# Autodesk Inventor assembly: CrutchCupHolder
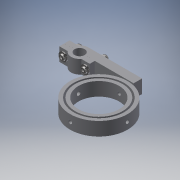
[picture p0: Inventor's stored thumbnail of the model, 180x180]
Saved by Autodesk Inventor 2017 SP1 (Build 210196100, 196)
## iProperties
Created: 2016-07-31
Part Number: CrutchCupHolder
Document SubType Name: Assembly
Designer: steele
Author: steele
## Documents named in this file (8)
- D:\snobotics\CAD-Development\robSteele\HouseProjects\CrutchProjects\CrutchCupHolder.iam
- D:\snobotics\CAD-Development\robSteele\HouseProjects\CrutchProjects\Innerring.ipt
- D:\snobotics\CAD-Development\robSteele\HouseProjects\CrutchProjects\outerRing.ipt
- D:\snobotics\CAD-Development\robSteele\HouseProjects\CrutchProjects\outerCrutchAttacement.ipt
- D:\snobotics\CAD-Development\robSteele\HouseProjects\CrutchProjects\innerCrutchAttacement.ipt
- D:\snobotics\CAD-Development\robSteele\HouseProjects\CrutchProjects\CrutchCupHolder\Design Accelerator\Bolted Connection1.iam
- D:\snobotics\CAD-Development\robSteele\HouseProjects\CrutchProjects\CrutchCupHolder\Design Accelerator\Bolted Connection2.iam
- D:\snobotics\CAD-Development\robSteele\HouseProjects\CrutchProjects\CrutchCupHolder\Design Accelerator\Clevis Pin Connection4.iam
## Components (7 placed, 6 different names)
1. Innerring:1 — Insert:1
2. outerRing:1 — Mate:8, Insert:1
3. outerCrutchAttacement:1 — Mate:1, Flush:1, Flush:2, Mate:9, Mate:10
4. innerCrutchAttacement:1 — Mate:1, Flush:1, Flush:2, Mate:2, Mate:3, Mate:4, Mate:5
5. Bolted Connection:1 [sub-assembly] — Mate:2, Mate:3
6. Bolted Connection:2 [sub-assembly] — Mate:4, Mate:5
7. Clevis Pin Connection:1 [sub-assembly] — Mate:8, Mate:9, Mate:10
## Relationships (11: Mate 8, Flush 2, Insert 1)
- Mate:1: outerCrutchAttacement:1 ↔ innerCrutchAttacement:1
- Flush:1: outerCrutchAttacement:1 ↔ innerCrutchAttacement:1
- Flush:2: outerCrutchAttacement:1 ↔ innerCrutchAttacement:1
- Mate:2: innerCrutchAttacement:1 ↔ Bolted Connection:1
- Mate:3: innerCrutchAttacement:1 ↔ Bolted Connection:1
- Mate:4: innerCrutchAttacement:1 ↔ Bolted Connection:2
- Mate:5: innerCrutchAttacement:1 ↔ Bolted Connection:2
- Mate:8: outerRing:1 ↔ Clevis Pin Connection:1
- Insert:1: Innerring:1 ↔ outerRing:1
- Mate:9: outerCrutchAttacement:1 ↔ Clevis Pin Connection:1
- Mate:10: outerCrutchAttacement:1 ↔ Clevis Pin Connection:1
